# Autodesk Inventor assembly: Regulator 1764
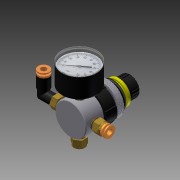
[picture p0: Inventor's stored thumbnail of the model, 180x180]
Saved by Autodesk Inventor 2011 (Build 150239000, 239)
## iProperties
Created: 2010-02-17
Part Number: Regulator 1764
Document SubType Name: Assembly
Designer: jgehrig
Author: jgehrig
## Documents named in this file (9)
- R:\CAD Archives\Pneumatics\Regulator 1764\Regulator 1764.iam
- R:\CAD Archives\Pneumatics\Regulator 1764\Regulator Base 1764.ipt
- R:\CAD Archives\Pneumatics\Regulator 1764\Regulator Middle 1764.ipt
- R:\CAD Archives\Pneumatics\Regulator 1764\PSI Gage 1764\PSI Gauge 1764.iam
- R:\CAD Archives\Pneumatics\Regulator 1764\Regulator Ring 1 1764.ipt
- R:\CAD Archives\Pneumatics\Regulator 1764\Regulator Ring 2 1764.ipt
- R:\CAD Archives\Pneumatics\Regulator 1764\Pneumatic Screw 1764\Pneumatic Screw 1764.iam
- R:\CAD Archives\Pneumatics\Regulator 1764\Pneumatics Bend Piece 1764\Pneumatic Bend Piece 1764.iam
- R:\CAD Archives\Pneumatics\Regulator 1764\Pneumatic Screw 1764\Pneumatic Screw Part 1 1764.ipt
## Components (8 placed, 8 different names)
1. Regulator Base 1764:1 — Insert:1, Mate:1, Tangent:1, Mate:2, Tangent:2, Mate:3, Tangent:3, Mate:4, Tangent:4
2. Regulator Middle 1764:1 — Insert:1, Insert:2, Insert:3, Angle:1
3. Regulator Ring 1 1764:1 — Insert:3
4. Regulator Ring 2 1764:1 — Insert:2
5. PSI Gauge 1764:1 [sub-assembly] — Mate:1, Tangent:1, Angle:1, Angle:2
6. Pneumatic Screw 1764:1 [sub-assembly] — Mate:2, Tangent:2
7. Pneumatic Bend Piece 1764:1 [sub-assembly] — Mate:3, Tangent:3, Angle:2
8. Pneumatic Screw Part 1 1764:1 — Mate:4, Tangent:4
## Relationships (13: Mate 4, Tangent 4, Insert 3, Angle 2)
- Insert:1: Regulator Base 1764:1 ↔ Regulator Middle 1764:1
- Insert:2: Regulator Middle 1764:1 ↔ Regulator Ring 2 1764:1
- Insert:3 (3.175 mm): Regulator Middle 1764:1 ↔ Regulator Ring 1 1764:1
- Mate:1: Regulator Base 1764:1 ↔ PSI Gauge 1764:1
- Tangent:1 (3.175 mm): Regulator Base 1764:1 ↔ PSI Gauge 1764:1
- Angle:1 (0 deg): Regulator Middle 1764:1 ↔ PSI Gauge 1764:1
- Mate:2: Regulator Base 1764:1 ↔ Pneumatic Screw 1764:1
- Tangent:2 (3.175 mm): Regulator Base 1764:1 ↔ Pneumatic Screw 1764:1
- Mate:3: Regulator Base 1764:1 ↔ Pneumatic Bend Piece 1764:1
- Tangent:3 (3.175 mm): Regulator Base 1764:1 ↔ Pneumatic Bend Piece 1764:1
- Angle:2 (0 deg): PSI Gauge 1764:1 ↔ Pneumatic Bend Piece 1764:1
- Mate:4: Regulator Base 1764:1 ↔ Pneumatic Screw Part 1 1764:1
- Tangent:4 (3.175 mm): Regulator Base 1764:1 ↔ Pneumatic Screw Part 1 1764:1
